# Autodesk Inventor assembly: both sides of drive
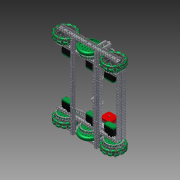
[picture p0: Inventor's stored thumbnail of the model, 180x180]
Saved by Autodesk Inventor 2014 SP1 (Build 180222100, 222)
## iProperties
Created: 2014-03-07
Part Number: both sides of drive
Document SubType Name: Assembly
Designer: Ryan
Author: Ryan
## Documents named in this file (7)
- C:\Users\Ryan\Desktop\sw\toss up 5th A bot\drive\both sides of drive.iam
- C:\Users\Ryan\Desktop\sw\toss up 5th A bot\drive\one side of drive.iam
- C:\Users\Ryan\Desktop\sw\lib\Aperture VEX CAD Library\Metal\L Bar\2 x 25.ipt
- C:\Users\Ryan\Desktop\sw\toss up 5th A bot\drive\1x1 tube.iam
- C:\Users\Ryan\Desktop\sw\toss up 5th A bot\drive\one side of drive_MIR.iam
- C:\Users\Ryan\Desktop\sw\toss up 5th A bot\drive\bump thing.iam
- C:\Users\Ryan\Desktop\sw\toss up 5th A bot\drive\hardstop.iam
## Components (10 placed, 6 different names)
1. one side of drive:1 [sub-assembly] — Mate:1, Flush:1, Flush:2, Mate:3, Flush:5, Flush:6, Mate:4, Flush:7, Flush:8, Mate:5, Flush:10, Flush:11
2. 2 x 25:1 — Mate:1, Flush:1, Flush:2, Mate:2, Flush:3, Flush:4, Flush:9
3. 2 x 25:2 — Mate:2, Flush:3, Flush:4
4. 1x1 tube:1 [sub-assembly] — Mate:3, Flush:5, Flush:6
5. 1x1 tube:2 [sub-assembly] — Mate:4, Flush:7, Flush:8
6. one side of drive_MIR:1 [sub-assembly]
7. 2 x 25:3 — Mate:5, Flush:10, Flush:11, Mate:6, Mate:7, Mate:8, Mate:9, Flush:12, Flush:13
8. bump thing:1 [sub-assembly] — Mate:6, Mate:7, Mate:8
9. hardstop:1 [sub-assembly] — Mate:9, Flush:12, Flush:13
10. hardstop:2 [sub-assembly]
## Component patterns: (2 elements, first: hardstop:1)
## Relationships (22: Flush 13, Mate 9)
- Mate:1 (1.5875 mm): one side of drive:1 ↔ 2 x 25:1
- Flush:1: one side of drive:1 ↔ 2 x 25:1
- Flush:2: one side of drive:1 ↔ 2 x 25:1
- Mate:2: 2 x 25:1 ↔ 2 x 25:2
- Flush:3: 2 x 25:1 ↔ 2 x 25:2
- Flush:4: 2 x 25:1 ↔ 2 x 25:2
- Mate:3: one side of drive:1 ↔ 1x1 tube:1
- Flush:5: one side of drive:1 ↔ 1x1 tube:1
- Flush:6: one side of drive:1 ↔ 1x1 tube:1
- Mate:4: one side of drive:1 ↔ 1x1 tube:2
- Flush:7: one side of drive:1 ↔ 1x1 tube:2
- Flush:8: one side of drive:1 ↔ 1x1 tube:2
- Flush:9 (-158.75 mm): 2 x 25:1
- Mate:5: one side of drive:1 ↔ 2 x 25:3
- Flush:10: one side of drive:1 ↔ 2 x 25:3
- Flush:11: one side of drive:1 ↔ 2 x 25:3
- Mate:6 (2.3114 mm): 2 x 25:3 ↔ bump thing:1
- Mate:7 (2.3114 mm): 2 x 25:3 ↔ bump thing:1
- Mate:8: 2 x 25:3 ↔ bump thing:1
- Mate:9: 2 x 25:3 ↔ hardstop:1
- Flush:12: 2 x 25:3 ↔ hardstop:1
- Flush:13: 2 x 25:3 ↔ hardstop:1
## Named parameters: q = 2.3114 mm
